# Autodesk Inventor assembly: КВ33.044.1000 - Блок управления
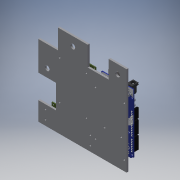
[picture p0: Inventor's stored thumbnail of the model, 180x180]
Saved by Autodesk Inventor 2019 (Build 230136000, 136)
## iProperties
Created: 2019-10-30
Part Number: КВ33.044.1000 - Блок управления
Material: Типовые
Document SubType Name: Assembly
Designer: Петров Иван
Author: Петров Иван
## Documents named in this file (5)
- E:\IVAN\Ivan_desktop\Kvantorium\Projects\optimal_gripper\hardware\КВ33.044.1000 - Блок управления.iam
- E:\IVAN\Ivan_desktop\Kvantorium\Projects\optimal_gripper\hardware\КВ33.044.1001 - Дно платы.ipt
- E:\IVAN\Ivan_desktop\Kvantorium\Projects\optimal_gripper\hardware\Стандартные изделия\Платформа Arduino MEGA 2560.ipt
- E:\IVAN\Ivan_desktop\Kvantorium\Projects\optimal_gripper\hardware\КВ33.044.1002 - Плата распределительная.ipt
- E:\IVAN\Ivan_desktop\Kvantorium\Projects\optimal_gripper\hardware\КВ33.044.1003 - Плата контроля сервомоторами.ipt
## Components (4 placed, 4 different names)
1. КВ33.044.1001 - Дно платы:1 — Совмещение:1, Совмещение:2, Совмещение:3, Совмещение:4, Совмещение:5, Совмещение:6, Совмещение:7, Совмещение:8, Совмещение:9
2. Платформа Arduino MEGA 2560:1 — Совмещение:1, Совмещение:2, Совмещение:3
3. КВ33.044.1002 - Плата распределительная:1 — Совмещение:4, Совмещение:5, Совмещение:6
4. КВ33.044.1003 - Плата контроля сервомоторами:1 — Совмещение:7, Совмещение:8, Совмещение:9
## Relationships (9: Mate 9)
- Совмещение:1 [Mate] (10 mm): КВ33.044.1001 - Дно платы:1 ↔ Платформа Arduino MEGA 2560:1
- Совмещение:2 [Mate]: КВ33.044.1001 - Дно платы:1 ↔ Платформа Arduino MEGA 2560:1
- Совмещение:3 [Mate]: КВ33.044.1001 - Дно платы:1 ↔ Платформа Arduino MEGA 2560:1
- Совмещение:4 [Mate] (10 mm): КВ33.044.1001 - Дно платы:1 ↔ КВ33.044.1002 - Плата распределительная:1
- Совмещение:5 [Mate]: КВ33.044.1001 - Дно платы:1 ↔ КВ33.044.1002 - Плата распределительная:1
- Совмещение:6 [Mate]: КВ33.044.1001 - Дно платы:1 ↔ КВ33.044.1002 - Плата распределительная:1
- Совмещение:7 [Mate] (10 mm): КВ33.044.1001 - Дно платы:1 ↔ КВ33.044.1003 - Плата контроля сервомоторами:1
- Совмещение:8 [Mate]: КВ33.044.1001 - Дно платы:1 ↔ КВ33.044.1003 - Плата контроля сервомоторами:1
- Совмещение:9 [Mate]: КВ33.044.1001 - Дно платы:1 ↔ КВ33.044.1003 - Плата контроля сервомоторами:1
